# Autodesk Inventor assembly: Нога левая в сборе 2_Зеркало
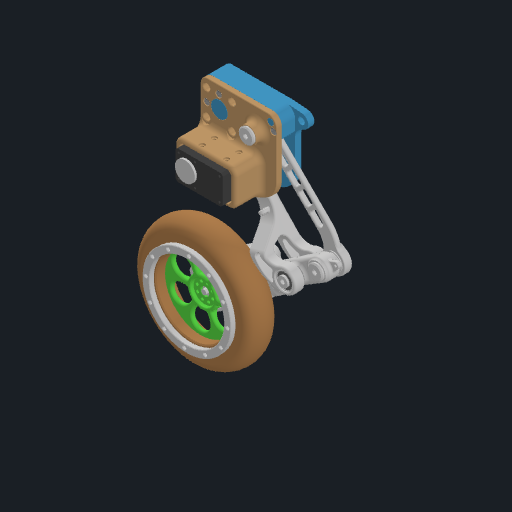
[picture p0: Inventor's stored thumbnail of the model, 512x512]
Saved by Autodesk Inventor 2025 (Build 290162010, 162A)
## iProperties
Created: 2024-06-21
Part Number: Нога левая в сборе 2_Зеркало
Document SubType Name: Assembly
Designer: Edward_Higgins
Author: Edward_Higgins
## Documents named in this file (13)
- D:\Users\Edward_Higgins\Desktop\ZAVOD\Робот Сколково\Нога левая в сборе 2_Зеркало.iam
- D:\Users\Edward_Higgins\Desktop\ZAVOD\Робот Сколково\Тяга передняя_Зеркало.ipt
- D:\Users\Edward_Higgins\Desktop\ZAVOD\Робот Сколково\DYNAMIXEL XM430-W350.ipt
- D:\Users\Edward_Higgins\Desktop\ZAVOD\Робот Сколково\Голень в сборе.iam
- D:\Users\Edward_Higgins\Desktop\ZAVOD\Робот Сколково\Подшипник.ipt
- D:\Users\Edward_Higgins\Desktop\ZAVOD\Робот Сколково\Стопорная шайба.ipt
- D:\Users\Edward_Higgins\Desktop\ZAVOD\Робот Сколково\Шайба.ipt
- D:\Users\Edward_Higgins\Desktop\ZAVOD\Робот Сколково\Ось односторонняя.ipt
- D:\Users\Edward_Higgins\Desktop\ZAVOD\Робот Сколково\Колесо 2 в сборе.iam
- D:\Users\Edward_Higgins\Desktop\ZAVOD\Робот Сколково\Корпус ноги в сборе_Зеркало.iam
- D:\Users\Edward_Higgins\Desktop\ZAVOD\Робот Сколково\Тяга задняя 2_Зеркало.ipt
- D:\Users\Edward_Higgins\Desktop\ZAVOD\Робот Сколково\Ось шарнира.ipt
- D:\Users\Edward_Higgins\Desktop\ZAVOD\Робот Сколково\Ось двусторонняя.ipt
## Components (19 placed, 12 different names)
1. Тяга передняя_Зеркало:1 — Совмещение:84, Совмещение:21, Совмещение:121, Совмещение:85, Совмещение:103, Совмещение:137, Совмещение:115, Совмещение:113, Совмещение:129, Совмещение:124
2. DYNAMIXEL XM430-W350:1 — Совмещение:84, Совмещение:21, Совмещение:104, Угол:1
3. Голень в сборе:1 [sub-assembly] — Совмещение:121, Совмещение:85, Совмещение:100, Совмещение:99, Совмещение:105, Совмещение:116, Совмещение:122
4. Подшипник:1 — Совмещение:91, Совмещение:90, Совмещение:93, Совмещение:92, Совмещение:110
5. Стопорная шайба:1 — Совмещение:91, Совмещение:90
6. Шайба:1 — Совмещение:96, Совмещение:94, Совмещение:109
7. Ось односторонняя:1 — Совмещение:96, Совмещение:94, Совмещение:93, Совмещение:92, Совмещение:108, Совмещение:107
8. Колесо 2 в сборе:1 [sub-assembly] — Совмещение:100, Совмещение:99
9. Корпус ноги в сборе_Зеркало:1 [sub-assembly] — Совмещение:109, Совмещение:108, Совмещение:107, Совмещение:104, Угол:1, Совмещение:103, Совмещение:102, Совмещение:101
10. Тяга задняя 2_Зеркало:1 — Совмещение:110, Совмещение:105, Совмещение:120, Совмещение:119
11. Ось шарнира:1 — Совмещение:137, Совмещение:115, Совмещение:113, Совмещение:136
12. Подшипник:2 — Совмещение:120, Совмещение:119, Совмещение:116, Совмещение:118, Совмещение:117
13. Стопорная шайба:2 — Совмещение:118, Совмещение:117
14. Подшипник:3 — Совмещение:129, Совмещение:131, Совмещение:130, Совмещение:128
15. Стопорная шайба:3 — Совмещение:131, Совмещение:130
16. Подшипник:4 — Совмещение:124, Совмещение:127, Совмещение:126, Совмещение:125, Совмещение:123
17. Стопорная шайба:4 — Совмещение:127, Совмещение:126
18. Ось двусторонняя:1 — Совмещение:128, Совмещение:125, Совмещение:123, Совмещение:122
19. Подшипник:5 — Совмещение:136
## Relationships (41: Mate 40, Angle 1)
- Совмещение:84 [Mate]: Тяга передняя_Зеркало:1 ↔ DYNAMIXEL XM430-W350:1
- Совмещение:21 [Mate]: Тяга передняя_Зеркало:1 ↔ DYNAMIXEL XM430-W350:1
- Совмещение:121 [Mate]: Тяга передняя_Зеркало:1 ↔ Голень в сборе:1
- Совмещение:85 [Mate]: Тяга передняя_Зеркало:1 ↔ Голень в сборе:1
- Совмещение:91 [Mate]: Подшипник:1 ↔ Стопорная шайба:1
- Совмещение:90 [Mate]: Подшипник:1 ↔ Стопорная шайба:1
- Совмещение:96 [Mate]: Шайба:1 ↔ Ось односторонняя:1
- Совмещение:94 [Mate]: Шайба:1 ↔ Ось односторонняя:1
- Совмещение:93 [Mate]: Подшипник:1 ↔ Ось односторонняя:1
- Совмещение:92 [Mate]: Подшипник:1 ↔ Ось односторонняя:1
- Совмещение:100 [Mate]: Голень в сборе:1 ↔ Колесо 2 в сборе:1
- Совмещение:99 [Mate]: Голень в сборе:1 ↔ Колесо 2 в сборе:1
- Совмещение:109 [Mate]: Шайба:1 ↔ Корпус ноги в сборе_Зеркало:1
- Совмещение:108 [Mate]: Ось односторонняя:1 ↔ Корпус ноги в сборе_Зеркало:1
- Совмещение:107 [Mate]: Ось односторонняя:1 ↔ Корпус ноги в сборе_Зеркало:1
- Совмещение:104 [Mate]: DYNAMIXEL XM430-W350:1 ↔ Корпус ноги в сборе_Зеркало:1
- Угол:1 [Angle] (0 deg): DYNAMIXEL XM430-W350:1 ↔ Корпус ноги в сборе_Зеркало:1
- Совмещение:103 [Mate]: Тяга передняя_Зеркало:1 ↔ Корпус ноги в сборе_Зеркало:1
- Совмещение:102 [Mate]: Корпус ноги в сборе_Зеркало:1
- Совмещение:101 [Mate]: Корпус ноги в сборе_Зеркало:1
- Совмещение:110 [Mate]: Подшипник:1 ↔ Тяга задняя 2_Зеркало:1
- Совмещение:105 [Mate]: Голень в сборе:1 ↔ Тяга задняя 2_Зеркало:1
- Совмещение:137 [Mate]: Тяга передняя_Зеркало:1 ↔ Ось шарнира:1
- Совмещение:115 [Mate]: Тяга передняя_Зеркало:1 ↔ Ось шарнира:1
- Совмещение:113 [Mate]: Тяга передняя_Зеркало:1 ↔ Ось шарнира:1
- Совмещение:120 [Mate]: Тяга задняя 2_Зеркало:1 ↔ Подшипник:2
- Совмещение:119 [Mate]: Тяга задняя 2_Зеркало:1 ↔ Подшипник:2
- Совмещение:116 [Mate]: Голень в сборе:1 ↔ Подшипник:2
- Совмещение:118 [Mate]: Подшипник:2 ↔ Стопорная шайба:2
- Совмещение:117 [Mate]: Подшипник:2 ↔ Стопорная шайба:2
- Совмещение:129 [Mate]: Тяга передняя_Зеркало:1 ↔ Подшипник:3
- Совмещение:131 [Mate]: Подшипник:3 ↔ Стопорная шайба:3
- Совмещение:130 [Mate]: Подшипник:3 ↔ Стопорная шайба:3
- Совмещение:124 [Mate]: Тяга передняя_Зеркало:1 ↔ Подшипник:4
- Совмещение:127 [Mate]: Подшипник:4 ↔ Стопорная шайба:4
- Совмещение:126 [Mate]: Подшипник:4 ↔ Стопорная шайба:4
- Совмещение:128 [Mate]: Подшипник:3 ↔ Ось двусторонняя:1
- Совмещение:125 [Mate]: Подшипник:4 ↔ Ось двусторонняя:1
- Совмещение:123 [Mate]: Подшипник:4 ↔ Ось двусторонняя:1
- Совмещение:122 [Mate]: Голень в сборе:1 ↔ Ось двусторонняя:1
- Совмещение:136 [Mate]: Ось шарнира:1 ↔ Подшипник:5
